# Autodesk Inventor assembly: omni_platforma
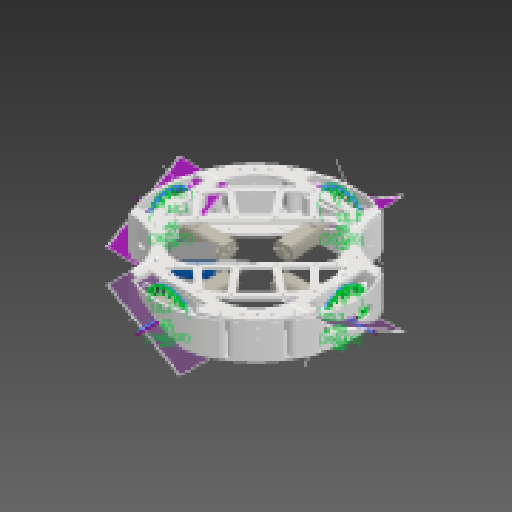
[picture p0: Inventor's stored thumbnail of the model, 512x512]
Saved by Autodesk Inventor 2023 (Build 270158000, 158)
## iProperties
Created: 2025-06-27
Part Number: omni_platforma
Document SubType Name: Assembly
Designer: daa
Author: daa
## Documents named in this file (13)
- C:\Users\daa\Documents\DASH_V2\omni_platforma\omni_platforma.iam
- C:\Users\daa\Documents\DASH_V2\omni_platforma\bottom.ipt
- C:\Users\daa\Documents\DASH_V2\omni_platforma\fastenin_motor.ipt
- C:\Users\daa\Documents\DASH_V2\omni_platforma\motor20.ipt
- C:\Users\daa\Documents\DASH_V2\omni_platforma\Wheel.iam
- C:\Users\daa\Documents\DASH_V2\omni_platforma\ball_solenoid.ipt
- C:\Users\daa\Documents\DASH_V2\omni_platforma\handle mount.ipt
- C:\Users\daa\Documents\DASH_V2\omni_platforma\protect.ipt
- C:\Users\daa\Documents\DASH_V2\omni_platforma\Деталь3.ipt
- C:\Users\daa\Documents\DASH_V2\omni_platforma\Solenoid.iam
- C:\Users\daa\Documents\DASH_V2\omni_platforma\top_v2.ipt
- C:\Users\daa\Documents\DASH_V2\omni_platforma\protect_2.ipt
- C:\Users\daa\Documents\DASH_V2\omni_platforma\ball_solenoid_v2.ipt
## Components (24 placed, 12 different names)
1. bottom:1 — С поворотом:1, С поворотом:4, С поворотом:6, С поворотом:8, С поворотом:13, С поворотом:15, С поворотом:16, С поворотом:18, С поворотом:20, С поворотом:21, С поворотом:24, С поворотом:25
2. fastenin_motor:1 — С поворотом:4, С поворотом:5
3. motor20:1 — С поворотом:2, С поворотом:3
4. Wheel:1 [sub-assembly] — С поворотом:11
5. fastenin_motor:2 — С поворотом:6, С поворотом:7
6. motor20:2 — С поворотом:7, С поворотом:11
7. Wheel:2 [sub-assembly] — С поворотом:10
8. fastenin_motor:3 — С поворотом:8, С поворотом:9
9. motor20:3 — С поворотом:9, С поворотом:12
10. Wheel:3 [sub-assembly] — С поворотом:12
11. fastenin_motor:4 — С поворотом:1, С поворотом:2
12. motor20:4 — С поворотом:5, С поворотом:10
13. Wheel:4 [sub-assembly] — С поворотом:3
14. ball_solenoid:1 — С поворотом:13, С поворотом:23
15. handle mount:1 — С поворотом:15
16. handle mount:2 — С поворотом:16
17. protect:2 — С поворотом:20
18. protect:3 — С поворотом:18
19. Деталь3:1 — С поворотом:21, С поворотом:22
20. Solenoid:1 [sub-assembly] — С поворотом:22
21. top_v2:1 — С поворотом:23
22. protect_2:1 — С поворотом:24
23. protect_2:2 — С поворотом:25
24. ball_solenoid_v2:1
## Relationships (22: RevoluteJoint 22)
- С поворотом:1 [RevoluteJoint]: bottom:1 ↔ fastenin_motor:4
- С поворотом:2 [RevoluteJoint]: motor20:1 ↔ fastenin_motor:4
- С поворотом:3 [RevoluteJoint] (-7 mm): motor20:1 ↔ Wheel:4
- С поворотом:4 [RevoluteJoint]: bottom:1 ↔ fastenin_motor:1
- С поворотом:5 [RevoluteJoint]: fastenin_motor:1 ↔ motor20:4
- С поворотом:6 [RevoluteJoint]: bottom:1 ↔ fastenin_motor:2
- С поворотом:7 [RevoluteJoint]: fastenin_motor:2 ↔ motor20:2
- С поворотом:8 [RevoluteJoint]: bottom:1 ↔ fastenin_motor:3
- С поворотом:9 [RevoluteJoint]: fastenin_motor:3 ↔ motor20:3
- С поворотом:10 [RevoluteJoint] (-7 mm): Wheel:2 ↔ motor20:4
- С поворотом:11 [RevoluteJoint] (-7 mm): Wheel:1 ↔ motor20:2
- С поворотом:12 [RevoluteJoint] (-7 mm): motor20:3 ↔ Wheel:3
- С поворотом:13 [RevoluteJoint]: bottom:1 ↔ ball_solenoid:1
- С поворотом:15 [RevoluteJoint]: bottom:1 ↔ handle mount:1
- С поворотом:16 [RevoluteJoint]: bottom:1 ↔ handle mount:2
- С поворотом:18 [RevoluteJoint]: bottom:1 ↔ protect:3
- С поворотом:20 [RevoluteJoint]: bottom:1 ↔ protect:2
- С поворотом:21 [RevoluteJoint]: bottom:1 ↔ Деталь3:1
- С поворотом:22 [RevoluteJoint]: Деталь3:1 ↔ Solenoid:1
- С поворотом:23 [RevoluteJoint]: ball_solenoid:1 ↔ top_v2:1
- С поворотом:24 [RevoluteJoint]: bottom:1 ↔ protect_2:1
- С поворотом:25 [RevoluteJoint]: bottom:1 ↔ protect_2:2
